# Autodesk Inventor assembly: Galileo Body
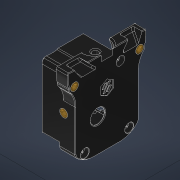
[picture p0: Inventor's stored thumbnail of the model, 180x180]
Saved by Autodesk Inventor 2022.2 (Build 262287010, 287A)
## iProperties
Created: 2022-03-15
Part Number: Galileo Body
Document SubType Name: Assembly
Designer: sleib
Author: sleib
## Documents named in this file (3)
- C:\Users\sleib\Projekte\Voron-2\CAD\Inventor\Galileo Clockwork\Galileo Body.iam
- C:\Users\sleib\Projekte\Voron-2\CAD\Inventor\Galileo Clockwork\Main Body Coupler.ipt
- C:\Users\sleib\Projekte\Voron-2\CAD\Inventor\M3 Threaded Insert.ipt
## Components (6 placed, 2 different names)
1. Main Body Coupler:1 — Passend:1, Passend:2, Passend:3, Passend:4, Fluchtend:1, Fluchtend:2, Fluchtend:3, Fluchtend:4, Passend:5, Fluchtend:5
2. M3 Threaded Insert:1 — Passend:1, Fluchtend:3
3. M3 Threaded Insert:2 — Passend:2, Fluchtend:4
4. M3 Threaded Insert:3 — Passend:3, Fluchtend:2
5. M3 Threaded Insert:4 — Passend:4, Fluchtend:1
6. M3 Threaded Insert:5 — Passend:5, Fluchtend:5
## Relationships (10: Mate 5, Flush 5)
- Passend:1 [Mate]: Main Body Coupler:1 ↔ M3 Threaded Insert:1
- Passend:2 [Mate]: Main Body Coupler:1 ↔ M3 Threaded Insert:2
- Passend:3 [Mate]: Main Body Coupler:1 ↔ M3 Threaded Insert:3
- Passend:4 [Mate]: Main Body Coupler:1 ↔ M3 Threaded Insert:4
- Fluchtend:1 [Flush]: Main Body Coupler:1 ↔ M3 Threaded Insert:4
- Fluchtend:2 [Flush]: Main Body Coupler:1 ↔ M3 Threaded Insert:3
- Fluchtend:3 [Flush]: Main Body Coupler:1 ↔ M3 Threaded Insert:1
- Fluchtend:4 [Flush]: Main Body Coupler:1 ↔ M3 Threaded Insert:2
- Passend:5 [Mate]: Main Body Coupler:1 ↔ M3 Threaded Insert:5
- Fluchtend:5 [Flush]: Main Body Coupler:1 ↔ M3 Threaded Insert:5
